# Autodesk Inventor assembly: Assembly1
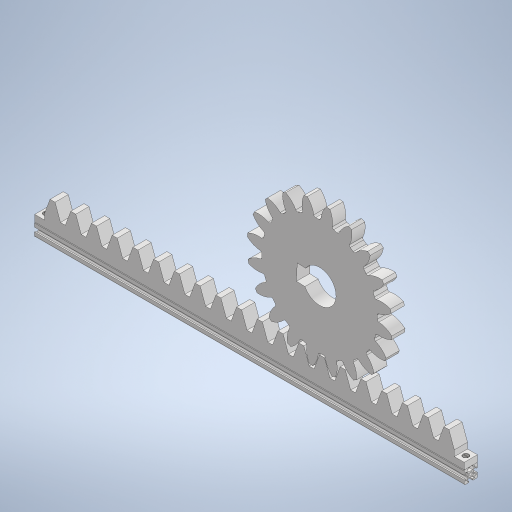
[picture p0: Inventor's stored thumbnail of the model, 512x512]
Saved by Autodesk Inventor 2023.2 (Build 272271030, 271C)
## iProperties
Created: 2023-03-04
Part Number: Assembly1
Document SubType Name: Assembly
Designer: Cris Pat
Author: Cris Pat
## Documents named in this file (6)
- C:\Users\Cris Pat\Desktop\U\Semestre 9\disenio e innovacion\CAD\Hbot\Assembly1.iam
- C:\Users\Cris Pat\Desktop\U\Semestre 9\disenio e innovacion\CAD\Hbot\piñon1.ipt
- C:\Users\Cris Pat\Desktop\U\Semestre 9\disenio e innovacion\CAD\Hbot\cremallera1.ipt
- C:\Users\Cris Pat\Documents\Inventor\Content Center Files\R2023\en-US\DIN 439-2\DIN 439 - M5 x 0.8.ipt
- C:\Users\Cris Pat\Desktop\U\Semestre 9\disenio e innovacion\CAD\Hbot\perfil_2020T.ipt
- C:\Users\Cris Pat\Documents\Inventor\Content Center Files\R2023\en-US\DIN 84\DIN 84 - M5 x 12.ipt
## Components (7 placed, 5 different names)
1. piñon1:1 — Mate:1, Mate:2, Flush:1, Rotation/Translation:1
2. cremallera1:1 — Flush:1, Flush:3, Rotation/Translation:1, Flush:4, Flush:5, Mate:3, Rotational:1, Rotational:3
3. DIN 84 - replaced by DIN EN ISO 1207 M5 x 12:1 — Rotational:1, Rotational:2
4. DIN 439-2 - replaced by DIN EN 24035/28675 M5:1 — Rotational:2
5. perfil_2020T:1 — Flush:4, Flush:5, Mate:3
6. DIN 84 - replaced by DIN EN ISO 1207 M5 x 12:2 — Rotational:3, Rigid:1
7. DIN 439-2 - replaced by DIN EN 24035/28675 M5:2 — Rigid:1
## Relationships (13: Flush 5, Mate 3, RevoluteJoint 3, RelateRotateTranslate 1, WeldJoint 1)
- Mate:1: piñon1:1
- Mate:2: piñon1:1
- Flush:1: piñon1:1 ↔ cremallera1:1
- Flush:2 (-100 mm)
- Flush:3 (12.5 mm): cremallera1:1
- Rotation/Translation:1 [RelateRotateTranslate] (628.32 mm): piñon1:1 ↔ cremallera1:1
- Flush:4: cremallera1:1 ↔ perfil_2020T:1
- Flush:5: cremallera1:1 ↔ perfil_2020T:1
- Mate:3: cremallera1:1 ↔ perfil_2020T:1
- Rotational:1 [RevoluteJoint]: cremallera1:1 ↔ DIN 84 - replaced by DIN EN ISO 1207 M5 x 12:1
- Rotational:2 [RevoluteJoint]: DIN 84 - replaced by DIN EN ISO 1207 M5 x 12:1 ↔ DIN 439-2 - replaced by DIN EN 24035/28675 M5:1
- Rotational:3 [RevoluteJoint]: cremallera1:1 ↔ DIN 84 - replaced by DIN EN ISO 1207 M5 x 12:2
- Rigid:1 [WeldJoint]: DIN 84 - replaced by DIN EN ISO 1207 M5 x 12:2 ↔ DIN 439-2 - replaced by DIN EN 24035/28675 M5:2
